# Autodesk Inventor assembly: Steering Electrical Assembly
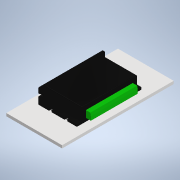
[picture p0: Inventor's stored thumbnail of the model, 180x180]
Saved by Autodesk Inventor 2020 (Build 240168000, 168)
## iProperties
Created: 2019-11-19
Part Number: Steering Electrical Assembly
Document SubType Name: Assembly
Designer: kylew
Author: kylew
## Documents named in this file (3)
- C:\Users\kylew\Desktop\Stepper Motor Mounting\Steering Electrical Assembly.iam
- C:\Users\kylew\Desktop\Stepper Motor Mounting\Aluminum_Heatsink_Base.ipt
- C:\Users\kylew\Desktop\Stepper Motor Mounting\CL57T_Stepper_Driver.ipt
## Components (2 placed, 2 different names)
1. Aluminum_Heatsink_Base:1 — Mate:1
2. CL57T_Stepper_Driver:1 — Mate:1
## Relationships (1: Mate 1)
- Mate:1: Aluminum_Heatsink_Base:1 ↔ CL57T_Stepper_Driver:1
